# Autodesk Inventor assembly: protoswitchboard
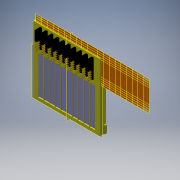
[picture p0: Inventor's stored thumbnail of the model, 180x180]
Saved by Autodesk Inventor 2017 (Build 210142000, 142)
## iProperties
Created: 2017-08-24
Part Number: protoswitchboard
Document SubType Name: Assembly
Designer: erwin
Author: erwin
## Documents named in this file (7)
- D:\GitHub\ProtoSwitchBoard\design\protoswitchboard.iam
- D:\GitHub\ProtoSwitchBoard\design\cover.ipt
- D:\GitHub\ProtoSwitchBoard\design\bottom.ipt
- D:\GitHub\ProtoSwitchBoard\documents\BusinessCard.ipt
- D:\GitHub\ProtoSwitchBoard\documents\Board.ipt
- D:\GitHub\ProtoSwitchBoard\documents\pinheader1.ipt
- D:\GitHub\ProtoSwitchBoard\documents\pinheader_female.ipt
## Components (104 placed, 6 different names)
1. cover:1 — Flush:1, Flush:2, Flush:3, Flush:4, Mate:1
2. bottom:1 — Flush:1, Flush:2
3. BusinessCard:1 — Flush:3, Flush:4
4. Board:1 — Mate:1, Flush:5, Flush:6, Flush:7, Flush:8, Flush:9, Flush:10
5. pinheader1:1 — Flush:5, Flush:6, Flush:7
6. pinheader1:2
7. pinheader1:3
8. pinheader1:4
9. pinheader1:5
10. pinheader1:6
11. pinheader1:7
12. pinheader1:8
13. pinheader1:9
14. pinheader1:10
15. pinheader1:11
16. pinheader1:12
17. pinheader1:13
18. pinheader1:14
19. pinheader1:15
20. pinheader1:16
21. pinheader1:17
22. pinheader1:18
23. pinheader1:19
24. pinheader1:20
25. pinheader1:21
26. pinheader1:22
27. pinheader1:23
28. pinheader1:24
29. pinheader1:25
30. pinheader1:26
31. pinheader1:27
32. pinheader1:28
33. pinheader1:29
34. pinheader1:30
35. pinheader1:31
36. pinheader1:32
37. pinheader1:33
38. pinheader1:34
39. pinheader1:35
40. pinheader1:36
41. pinheader1:37
42. pinheader1:38
43. pinheader1:39
44. pinheader1:40
45. pinheader1:41
46. pinheader1:42
47. pinheader1:43
48. pinheader1:44
49. pinheader1:45
50. pinheader1:46
51. pinheader1:47
52. pinheader1:48
53. pinheader1:49
54. pinheader1:50
55. pinheader_female:1 — Flush:8, Flush:9, Flush:10
56. pinheader_female:2
57. pinheader_female:3
58. pinheader_female:4
59. pinheader_female:5
60. pinheader_female:6
61. pinheader_female:7
62. pinheader_female:8
63. pinheader_female:9
64. pinheader_female:10
65. pinheader_female:11
66. pinheader_female:12
67. pinheader_female:13
68. pinheader_female:14
69. pinheader_female:15
70. pinheader_female:16
71. pinheader_female:17
72. pinheader_female:18
73. pinheader_female:19
74. pinheader_female:20
75. pinheader_female:21
76. pinheader_female:22
77. pinheader_female:23
78. pinheader_female:24
79. pinheader_female:25
80. pinheader_female:26
81. pinheader_female:27
82. pinheader_female:28
83. pinheader_female:29
84. pinheader_female:30
85. pinheader_female:31
86. pinheader_female:32
87. pinheader_female:33
88. pinheader_female:34
89. pinheader_female:35
90. pinheader_female:36
91. pinheader_female:37
92. pinheader_female:38
93. pinheader_female:39
94. pinheader_female:40
95. pinheader_female:41
96. pinheader_female:42
97. pinheader_female:43
98. pinheader_female:44
99. pinheader_female:45
100. pinheader_female:46
101. pinheader_female:47
102. pinheader_female:48
103. pinheader_female:49
104. pinheader_female:50
## Component patterns: (50 elements, first: pinheader1:1), (50 elements, first: pinheader_female:1)
## Relationships (11: Flush 10, Mate 1)
- Flush:1: cover:1 ↔ bottom:1
- Flush:2: cover:1 ↔ bottom:1
- Flush:3: cover:1 ↔ BusinessCard:1
- Flush:4: cover:1 ↔ BusinessCard:1
- Mate:1: cover:1 ↔ Board:1
- Flush:5: Board:1 ↔ pinheader1:1
- Flush:6: Board:1 ↔ pinheader1:1
- Flush:7: Board:1 ↔ pinheader1:1
- Flush:8: Board:1 ↔ pinheader_female:1
- Flush:9: Board:1 ↔ pinheader_female:1
- Flush:10: Board:1 ↔ pinheader_female:1
